# Autodesk Inventor assembly: boardC
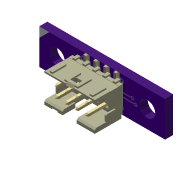
[picture p0: Inventor's stored thumbnail of the model, 180x180]
Saved by Autodesk Inventor 2017 (Build 210142000, 142)
## iProperties
Created: 2016-02-15
Part Number: boardC
Document SubType Name: Assembly
Designer: sawai
Author: sawai
## Documents named in this file (5)
- C:\Users\sawaiz\oneDrive\projects\mppcSensor\cad\sensorBoardC\boardC.iam
- C:\Users\sawaiz\oneDrive\projects\mppcSensor\cad\sensorBoardC\boardC.ipt
- C:\Users\sawaiz\oneDrive\projects\mppcSensor\cad\electronics\capacitor\capacitor-0603.ipt
- C:\Users\sawaiz\oneDrive\projects\mppcSensor\cad\electronics\capacitor.ipt
- C:\Users\sawaiz\oneDrive\projects\mppcSensor\cad\electronics\s98424-x52-08LF-clipped.ipt
## Components (4 placed, 3 different names)
1. boardC:1 — Mate:1, Mate:2, Flush:3
2. capacitor-0603:1 — Flush:1, Flush:2, Mate:1
3. capacitor-0603:2 — Flush:1, Flush:2
4. s98424-x52-08LF-clipped:1 — Mate:2, Flush:3
## Relationships (5: Flush 3, Mate 2)
- Flush:1: capacitor-0603:1 ↔ capacitor-0603:2
- Flush:2: capacitor-0603:1 ↔ capacitor-0603:2
- Mate:1: boardC:1 ↔ capacitor-0603:1
- Mate:2: boardC:1 ↔ s98424-x52-08LF-clipped:1
- Flush:3: boardC:1 ↔ s98424-x52-08LF-clipped:1
